# Autodesk Inventor assembly: test-model-SPG27
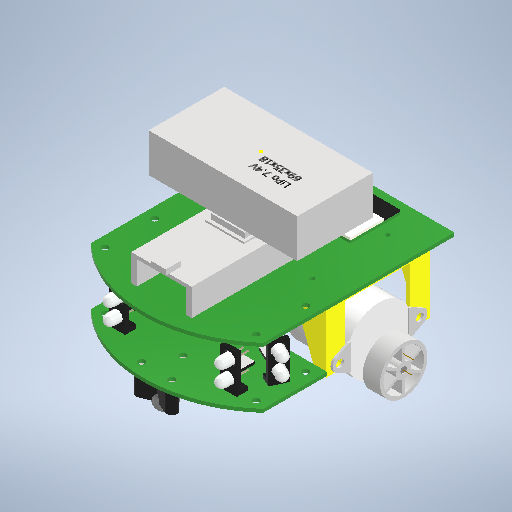
[picture p0: Inventor's stored thumbnail of the model, 512x512]
Saved by Autodesk Inventor 2025.3 (Build 293356000, 356)
## iProperties
Created: 2025-08-17
Part Number: test-model-SPG27
Document SubType Name: Assembly
Designer: daisuke
Author: daisuke
## Documents named in this file (11)
- G:\マイドライブ\project\micro-mouse\3D-Model\test-model-SPG27.iam
- G:\マイドライブ\project\micro-mouse\3D-Model\BaseBoard-SPG27.ipt
- G:\マイドライブ\project\micro-mouse\3D-Model\SPG27_asm.iam
- G:\マイドライブ\project\micro-mouse\3D-Model\Wheel-D22A.ipt
- G:\マイドライブ\project\micro-mouse\3D-Model\SensorBoard-SPG27.ipt
- G:\マイドライブ\project\micro-mouse\3D-Model\BallCaster-H16.ipt
- G:\マイドライブ\project\micro-mouse\3D-Model\Ground.ipt
- G:\マイドライブ\project\micro-mouse\3D-Model\ESP32-DevKitC.ipt
- G:\マイドライブ\project\micro-mouse\3D-Model\Photo-Sensor.iam
- G:\マイドライブ\project\micro-mouse\3D-Model\AQM1602Y.ipt
- G:\マイドライブ\project\micro-mouse\3D-Model\LiPo-7.4V-69x35x18.ipt
## Components (15 placed, 10 different names)
1. BaseBoard-SPG27:1 — メイト:1, メイト:2, メイト:3, メイト:4, メイト:5, メイト:6, メイト:12, メイト:13, メイト:15, メイト:20
2. SPG27_asm:1 [sub-assembly] — メイト:1, メイト:2, メイト:3, メイト:7, フラッシュ:1, メイト:14
3. SPG27_asm:2 [sub-assembly] — メイト:4, メイト:5, メイト:6, メイト:8, フラッシュ:2
4. Wheel-D22A:1 — メイト:7, フラッシュ:1
5. Wheel-D22A:2 — メイト:8, フラッシュ:2
6. SensorBoard-SPG27:1 — メイト:9, メイト:10, メイト:11, メイト:12, メイト:13, メイト:16, メイト:17, メイト:18, メイト:19
7. BallCaster-H16:1 — メイト:9, メイト:10, メイト:11, 正接:1
8. Ground:1 — メイト:14, 正接:1
9. ESP32-DevKitC:1 — メイト:15
10. Photo-Sensor:1 [sub-assembly] — メイト:17
11. Photo-Sensor:2 [sub-assembly] — メイト:18
12. Photo-Sensor:3 [sub-assembly] — メイト:16
13. Photo-Sensor:4 [sub-assembly] — メイト:19
14. AQM1602Y:1 — メイト:20
15. LiPo-7.4V-69x35x18:1
## Relationships (23: Mate 20, Flush 2, Tangent 1)
- メイト:1 [Mate]: BaseBoard-SPG27:1 ↔ SPG27_asm:1
- メイト:2 [Mate]: BaseBoard-SPG27:1 ↔ SPG27_asm:1
- メイト:3 [Mate]: BaseBoard-SPG27:1 ↔ SPG27_asm:1
- メイト:4 [Mate]: BaseBoard-SPG27:1 ↔ SPG27_asm:2
- メイト:5 [Mate]: BaseBoard-SPG27:1 ↔ SPG27_asm:2
- メイト:6 [Mate]: BaseBoard-SPG27:1 ↔ SPG27_asm:2
- メイト:7 [Mate]: SPG27_asm:1 ↔ Wheel-D22A:1
- フラッシュ:1 [Flush]: SPG27_asm:1 ↔ Wheel-D22A:1
- メイト:8 [Mate]: SPG27_asm:2 ↔ Wheel-D22A:2
- フラッシュ:2 [Flush]: SPG27_asm:2 ↔ Wheel-D22A:2
- メイト:9 [Mate]: SensorBoard-SPG27:1 ↔ BallCaster-H16:1
- メイト:10 [Mate]: SensorBoard-SPG27:1 ↔ BallCaster-H16:1
- メイト:11 [Mate]: SensorBoard-SPG27:1 ↔ BallCaster-H16:1
- メイト:12 [Mate]: BaseBoard-SPG27:1 ↔ SensorBoard-SPG27:1
- メイト:13 [Mate]: BaseBoard-SPG27:1 ↔ SensorBoard-SPG27:1
- メイト:14 [Mate] (14 mm): SPG27_asm:1 ↔ Ground:1
- 正接:1 [Tangent]: BallCaster-H16:1 ↔ Ground:1
- メイト:15 [Mate]: BaseBoard-SPG27:1 ↔ ESP32-DevKitC:1
- メイト:16 [Mate]: SensorBoard-SPG27:1 ↔ Photo-Sensor:3
- メイト:17 [Mate]: SensorBoard-SPG27:1 ↔ Photo-Sensor:1
- メイト:18 [Mate]: SensorBoard-SPG27:1 ↔ Photo-Sensor:2
- メイト:19 [Mate]: SensorBoard-SPG27:1 ↔ Photo-Sensor:4
- メイト:20 [Mate]: BaseBoard-SPG27:1 ↔ AQM1602Y:1
